# Autodesk Inventor assembly: encoderDiscAssembly
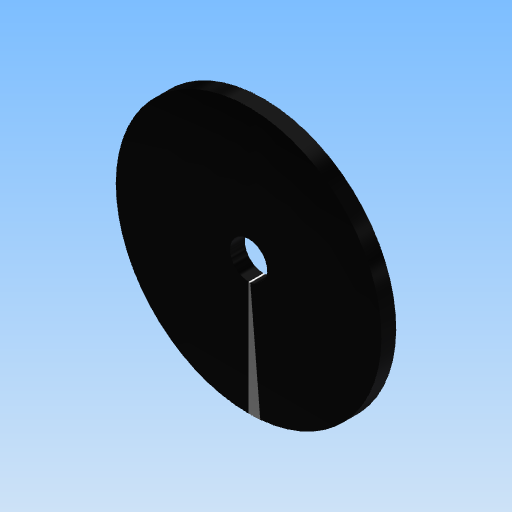
[picture p0: Inventor's stored thumbnail of the model, 512x512]
Saved by Autodesk Inventor 2017 (Build 210142000, 142)
## iProperties
Created: 2016-12-12
Part Number: encoderDiscAssembly
Document SubType Name: Assembly
Designer: techn
Author: techn
## Documents named in this file (3)
- D:\OneDrive\Documents\Other Projects\Submarine\CAD\aft\encoder\encoderDiscAssembly.iam
- D:\OneDrive\Documents\Other Projects\Submarine\CAD\aft\encoder\encoderDisc.ipt
- D:\OneDrive\Documents\Other Projects\Submarine\CAD\aft\encoder\encoderDiscNotch.ipt
## Components (2 placed, 2 different names)
1. encoderDisc:1 — Mate:1, Flush:1, Mate:2
2. encoderDiscNotch:1 — Mate:1, Flush:1, Mate:2
## Relationships (3: Mate 2, Flush 1)
- Mate:1: encoderDisc:1 ↔ encoderDiscNotch:1
- Flush:1: encoderDisc:1 ↔ encoderDiscNotch:1
- Mate:2: encoderDisc:1 ↔ encoderDiscNotch:1
